# Autodesk Inventor assembly: FirstAssembly
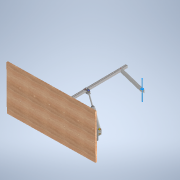
[picture p0: Inventor's stored thumbnail of the model, 180x180]
Saved by Autodesk Inventor 2022 (Build 260153000, 153)
## iProperties
Created: 2022-04-08
Part Number: FirstAssembly
Document SubType Name: Assembly
Designer: Patrick
Author: Patrick
## Documents named in this file (21)
- C:\Users\patri\OneDrive - Syddansk Universitet\2. Semester Master\Mekaniske Elementer\Mini Project\FirstAssembly.iam
- C:\Users\patri\OneDrive - Syddansk Universitet\2. Semester Master\Mekaniske Elementer\Mini Project\2020-10-23\Workspaces\Workspace\IMS-10-001.ipt
- C:\Users\patri\OneDrive - Syddansk Universitet\2. Semester Master\Mekaniske Elementer\Mini Project\2020-10-23\Workspaces\Workspace\IMS-00-003.ipt
- C:\Users\patri\OneDrive - Syddansk Universitet\2. Semester Master\Mekaniske Elementer\Mini Project\2020-10-23\Workspaces\Workspace\IMS-10-002.ipt
- C:\Users\patri\OneDrive - Syddansk Universitet\2. Semester Master\Mekaniske Elementer\Mini Project\2020-10-23\Workspaces\Workspace\Beslag_til_stempel'.iam
- C:\Users\patri\OneDrive - Syddansk Universitet\2. Semester Master\Mekaniske Elementer\Mini Project\2020-10-23\Workspaces\Workspace\Bushing_stempel.ipt
- C:\Users\patri\OneDrive - Syddansk Universitet\2. Semester Master\Mekaniske Elementer\Mini Project\2020-10-23\Workspaces\Workspace\Shatf_piston.ipt
- C:\Users\patri\OneDrive - Syddansk Universitet\2. Semester Master\Mekaniske Elementer\Mini Project\Beam.iam
- C:\Users\patri\OneDrive - Syddansk Universitet\2. Semester Master\Mekaniske Elementer\Mini Project\2020-10-23\Workspaces\Workspace\Bushing_beam.ipt
- C:\Users\patri\OneDrive - Syddansk Universitet\2. Semester Master\Mekaniske Elementer\Mini Project\2020-10-23\Workspaces\Workspace\193993 DSNU-40-300-P---(A---00--0-KS).ipt
- C:\Users\patri\OneDrive - Syddansk Universitet\2. Semester Master\Mekaniske Elementer\Mini Project\2020-10-23\Workspaces\Workspace\193993 DSNU-40-300-P---(A----0-ZR).ipt
- C:\Users\patri\OneDrive - Syddansk Universitet\2. Semester Master\Mekaniske Elementer\Mini Project\2020-10-23\Workspaces\Workspace\IMS-01-001.ipt
- C:\Users\patri\OneDrive - Syddansk Universitet\2. Semester Master\Mekaniske Elementer\Mini Project\2020-10-23\Workspaces\Workspace\beslag_stempel_stang.ipt
- C:\Users\patri\OneDrive - Syddansk Universitet\2. Semester Master\Mekaniske Elementer\Mini Project\2020-10-23\Workspaces\Workspace\Skive_stempel_stang.ipt
- C:\Users\patri\OneDrive - Syddansk Universitet\2. Semester Master\Mekaniske Elementer\Mini Project\2020-10-23\Workspaces\Workspace\pin_stempel_stang.ipt
- C:\Users\patri\OneDrive - Syddansk Universitet\2. Semester Master\Mekaniske Elementer\Mini Project\2020-10-23\Workspaces\Workspace\Exstra håndtag.iam
- C:\Users\patri\OneDrive - Syddansk Universitet\2. Semester Master\Mekaniske Elementer\Mini Project\2020-10-23\Workspaces\Workspace\Handle.ipt
- C:\Users\patri\OneDrive - Syddansk Universitet\2. Semester Master\Mekaniske Elementer\Mini Project\2020-10-23\Libraries\Content Center Files\en-US\ANSI B 27.7M(2)\ANSI B 27.7M - 3AMI-18.ipt
- C:\Users\patri\OneDrive - Syddansk Universitet\2. Semester Master\Mekaniske Elementer\Mini Project\2020-10-23\Workspaces\Workspace\Pin.ipt
- C:\Users\patri\OneDrive - Syddansk Universitet\2. Semester Master\Mekaniske Elementer\Mini Project\2020-10-23\Workspaces\Workspace\Pin til stang.ipt
- C:\Users\patri\OneDrive - Syddansk Universitet\2. Semester Master\Mekaniske Elementer\Mini Project\2020-10-23\Libraries\Content Center Files\en-US\ANSI B 27.7M(2)\ANSI B 27.7M - 3AMI-12.ipt
## Components (38 placed, 20 different names)
1. ClampOnBoard — Rigid:2, Rigid:4
2. BaseBoard — Rigid:2
3. ThreadsBaseBoard — Rigid:4, Mate:1, Mate:2, Mate:3, Rigid:8
4. Beslag_til_stempel':1 [sub-assembly] — Rotational:3, Rotational:4, Rigid:8
5. Bushing_stempel:1 — Rotational:4, Rigid:6
6. Bushing_stempel:2 — Rotational:3
7. Shatf_piston:1 — Rigid:6, Rotational:24, Rotational:42, Rotational:43
8. Beslag_til_stempel':2 [sub-assembly] — Mate:1, Mate:2, Rotational:6, Rotational:7, Mate:3
9. Bushing_beam:1 — Rotational:7, Rotational:9
10. Bushing_beam:2 — Rotational:6, Cylindrical:3
11. Shatf_piston:2 — Rotational:9, Rotational:44, Rotational:45
12. 193993 DSNU-40-300-P---(A---00--0-KS):1 — Rigid:11, Cylindrical:1
13. 193993 DSNU-40-300-P---(A----0-ZR):1 — Rotational:24, Cylindrical:1
14. beslag_stempel_stang:1 — Rigid:9, Rigid:10, Cylindrical:2, Cylindrical:4, Mate:5, Cylindrical:5, Rotational:32, Rotational:33
15. Skive_stempel_stang:1 — Rigid:9
16. Skive_stempel_stang:2 — Rigid:10
17. pin_stempel_stang:1 — Rotational:25, Cylindrical:2, Rotational:38, Rotational:39
18. IMS-01-001:1 — Rigid:11, Rotational:25
19. pin_stempel_stang:2 — Cylindrical:5
20. Beam:1 [sub-assembly] — Cylindrical:3, Cylindrical:4, Mate:5, Rotational:29
21. Handle:1 — Rotational:30, Cylindrical:6
22. ANSI B 27.7M 3AMI-18:1 — Rotational:38
23. ANSI B 27.7M 3AMI-18:2 — Rotational:39
24. Exstra håndtag:1 [sub-assembly] — Rotational:29, Rotational:30, Rotational:31
25. Pin:1 — Cylindrical:6
26. Pin til stang:1 — Rotational:31, Rotational:34, Rotational:35
27. Pin til stang:2 — Rotational:32, Rotational:36, Rotational:40
28. Pin til stang:3 — Rotational:33, Rotational:37, Rotational:41
29. ANSI B 27.7M 3AMI-12:1 — Rotational:37
30. ANSI B 27.7M 3AMI-12:2 — Rotational:36
31. ANSI B 27.7M 3AMI-12:3 — Rotational:41
32. ANSI B 27.7M 3AMI-12:4 — Rotational:40
33. ANSI B 27.7M 3AMI-12:5 — Rotational:34
34. ANSI B 27.7M 3AMI-12:6 — Rotational:35
35. ANSI B 27.7M 3AMI-12:7 — Rotational:45
36. ANSI B 27.7M 3AMI-12:8 — Rotational:44
37. ANSI B 27.7M 3AMI-12:9 — Rotational:42
38. ANSI B 27.7M 3AMI-12:10 — Rotational:43
## Relationships (41: RevoluteJoint 24, WeldJoint 7, CylindricalJoint 6, Mate 4)
- Rigid:2 [WeldJoint]: ClampOnBoard ↔ BaseBoard
- Rigid:4 [WeldJoint]: ClampOnBoard ↔ ThreadsBaseBoard
- Rotational:3 [RevoluteJoint]: Beslag_til_stempel':1 ↔ Bushing_stempel:2
- Rotational:4 [RevoluteJoint]: Beslag_til_stempel':1 ↔ Bushing_stempel:1
- Rigid:6 [WeldJoint]: Bushing_stempel:1 ↔ Shatf_piston:1
- Mate:1: ThreadsBaseBoard ↔ Beslag_til_stempel':2
- Mate:2: ThreadsBaseBoard ↔ Beslag_til_stempel':2
- Rotational:6 [RevoluteJoint]: Beslag_til_stempel':2 ↔ Bushing_beam:2
- Rotational:7 [RevoluteJoint]: Beslag_til_stempel':2 ↔ Bushing_beam:1
- Mate:3: ThreadsBaseBoard ↔ Beslag_til_stempel':2
- Rotational:9 [RevoluteJoint]: Bushing_beam:1 ↔ Shatf_piston:2
- Rigid:8 [WeldJoint]: ThreadsBaseBoard ↔ Beslag_til_stempel':1
- Rigid:9 [WeldJoint]: beslag_stempel_stang:1 ↔ Skive_stempel_stang:1
- Rigid:10 [WeldJoint]: beslag_stempel_stang:1 ↔ Skive_stempel_stang:2
- Rotational:24 [RevoluteJoint]: Shatf_piston:1 ↔ 193993 DSNU-40-300-P---(A----0-ZR):1
- Rigid:11 [WeldJoint]: 193993 DSNU-40-300-P---(A---00--0-KS):1 ↔ IMS-01-001:1
- Cylindrical:1: 193993 DSNU-40-300-P---(A---00--0-KS):1 ↔ 193993 DSNU-40-300-P---(A----0-ZR):1
- Rotational:25 [RevoluteJoint]: pin_stempel_stang:1 ↔ IMS-01-001:1
- Cylindrical:2: beslag_stempel_stang:1 ↔ pin_stempel_stang:1
- Cylindrical:3: Bushing_beam:2 ↔ Beam:1
- Cylindrical:4: beslag_stempel_stang:1 ↔ Beam:1
- Mate:5: beslag_stempel_stang:1 ↔ Beam:1
- Cylindrical:5: beslag_stempel_stang:1 ↔ pin_stempel_stang:2
- Rotational:29 [RevoluteJoint]: Beam:1 ↔ Exstra håndtag:1
- Rotational:30 [RevoluteJoint]: Handle:1 ↔ Exstra håndtag:1
- Cylindrical:6: Handle:1 ↔ Pin:1
- Rotational:31 [RevoluteJoint]: Exstra håndtag:1 ↔ Pin til stang:1
- Rotational:32 [RevoluteJoint]: beslag_stempel_stang:1 ↔ Pin til stang:2
- Rotational:33 [RevoluteJoint]: beslag_stempel_stang:1 ↔ Pin til stang:3
- Rotational:34 [RevoluteJoint]: Pin til stang:1 ↔ ANSI B 27.7M 3AMI-12:5
- Rotational:35 [RevoluteJoint]: Pin til stang:1 ↔ ANSI B 27.7M 3AMI-12:6
- Rotational:36 [RevoluteJoint]: Pin til stang:2 ↔ ANSI B 27.7M 3AMI-12:2
- Rotational:37 [RevoluteJoint]: Pin til stang:3 ↔ ANSI B 27.7M 3AMI-12:1
- Rotational:38 [RevoluteJoint]: pin_stempel_stang:1 ↔ ANSI B 27.7M 3AMI-18:1
- Rotational:39 [RevoluteJoint]: pin_stempel_stang:1 ↔ ANSI B 27.7M 3AMI-18:2
- Rotational:40 [RevoluteJoint]: Pin til stang:2 ↔ ANSI B 27.7M 3AMI-12:4
- Rotational:41 [RevoluteJoint]: Pin til stang:3 ↔ ANSI B 27.7M 3AMI-12:3
- Rotational:42 [RevoluteJoint]: Shatf_piston:1 ↔ ANSI B 27.7M 3AMI-12:9
- Rotational:43 [RevoluteJoint]: Shatf_piston:1 ↔ ANSI B 27.7M 3AMI-12:10
- Rotational:44 [RevoluteJoint]: Shatf_piston:2 ↔ ANSI B 27.7M 3AMI-12:8
- Rotational:45 [RevoluteJoint]: Shatf_piston:2 ↔ ANSI B 27.7M 3AMI-12:7
